# Autodesk Inventor assembly: ax4
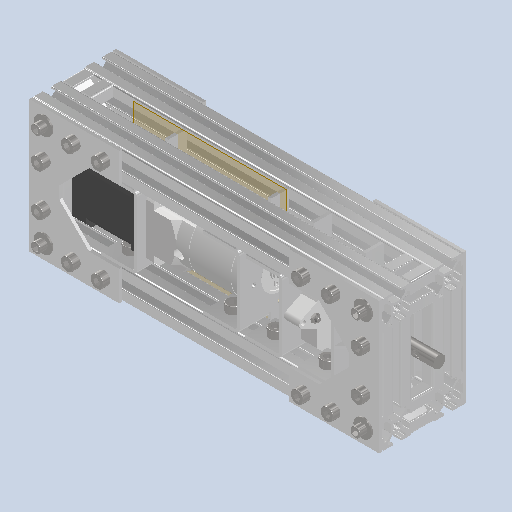
[picture p0: Inventor's stored thumbnail of the model, 512x512]
Saved by Autodesk Inventor 2024 (Build 280153000, 153)
## iProperties
Created: 2025-12-19
Part Number: ax4
Document SubType Name: Assembly
Designer: schar
Author: schar
## Documents named in this file (9)
- C:\Users\schar\Desktop\projectBlueprint\AMSTS\hardware\ax4.iam
- C:\Users\schar\Desktop\projectBlueprint\AMSTS\hardware\4x2020_in.iam
- C:\Users\schar\Desktop\projectBlueprint\AMSTS\hardware\4x2020_ax4.ipt
- C:\Users\schar\Desktop\projectBlueprint\AMSTS\hardware\2020_4x2020_hz.ipt
- C:\Users\schar\Desktop\projectBlueprint\AMSTS\hardware\2020_4x2020_ve.ipt
- C:\Users\schar\Desktop\projectBlueprint\AMSTS\hardware\Connect_u2020_asm.iam
- C:\Users\schar\Desktop\projectBlueprint\AMSTS\hardware\m4x70_example.ipt
- C:\Users\schar\Documents\Inventor\Content Center Files\R2024\en-US\DIN 9021\DIN 9021 - 4,3.ipt
- C:\Users\schar\Documents\Inventor\Content Center Files\R2024\en-US\ANSI B18.2.4.2M\ANSI B18.2.4.2M - M4x0,7 - 7.ipt
## Components (33 placed, 8 different names)
1. 4x2020_ax4:1 — Mate:1, Mate:2, Mate:3, Flush:1, Mate:4, Flush:2, Flush:4, Flush:8, Flush:10, Flush:13, Mate:12, Flush:17, Flush:18, Mate:15, Flush:23, Flush:24, Flush:28, Flush:31
2. 4x2020_ax4:2 — Mate:5, Flush:3, Flush:4, Flush:6, Mate:8, Flush:9, Mate:10, Flush:14, Mate:13, Flush:19, Flush:20, Mate:14, Flush:21, Flush:22, Mate:16, Flush:30
3. 4x2020_ax4:3 — Flush:7, Mate:7, Flush:8, Flush:11, Flush:12, Mate:11, Flush:15
4. 4x2020_ax4:4 — Mate:6, Flush:5, Flush:6, Mate:9, Flush:16, Flush:25, Flush:26
5. 4x2020_in:1 [sub-assembly] — Flush:1, Mate:4, Flush:2, Mate:5, Flush:3, Mate:6, Flush:5, Flush:7, Mate:7
6. 2020_4x2020_hz:1 — Mate:11, Flush:15, Flush:16
7. 2020_4x2020_hz:2 — Mate:10, Flush:13, Flush:14
8. 2020_4x2020_hz:3 — Mate:9, Flush:11, Flush:12
9. 2020_4x2020_hz:4 — Mate:8, Flush:9, Flush:10
10. 2020_4x2020_ve:1 — Mate:13, Flush:19, Flush:20, Flush:29, Mate:18
11. 2020_4x2020_ve:2 — Mate:12, Flush:17, Flush:18, Mate:19, Flush:32
12. 2020_4x2020_ve:3 — Mate:14, Flush:21, Flush:22
13. 2020_4x2020_ve:4 — Mate:15, Flush:23, Flush:24, Mate:17, Flush:27
14. Connect_u2020_asm:1 [sub-assembly] — Flush:25, Mate:16, Flush:26, Mate:22, Mate:23, Mate:24, Mate:25, Mate:40, Mate:42
15. Connect_u2020_asm:2 [sub-assembly] — Mate:17, Flush:27, Flush:28, Mate:20, Mate:21, Mate:26, Mate:27
16. Connect_u2020_asm:3 [sub-assembly] — Mate:19, Flush:31, Flush:32, Mate:28, Mate:29, Mate:30, Mate:31
17. Connect_u2020_asm:4 [sub-assembly] — Flush:29, Flush:30, Mate:18, Mate:32, Mate:33, Mate:34, Mate:35, Mate:36, Mate:38
18. m4x70_example:1 — Mate:42, Mate:43, Mate:48
19. m4x70_example:2 — Mate:40, Mate:41, Mate:50
20. m4x70_example:3 — Mate:38, Mate:39, Mate:46
21. m4x70_example:4 — Mate:36, Mate:37, Mate:44
22. DIN 9021 4,3:1 — Mate:32, Mate:35, Mate:37
23. DIN 9021 4,3:2 — Mate:24, Mate:25, Mate:43
24. DIN 9021 4,3:3 — Mate:22, Mate:23, Mate:41
25. DIN 9021 4,3:4 — Mate:33, Mate:34, Mate:39
26. DIN 9021 4,3:5 — Mate:20, Mate:21, Mate:51
27. DIN 9021 4,3:6 — Mate:26, Mate:27, Mate:49
28. DIN 9021 4,3:7 — Mate:30, Mate:31, Mate:45
29. DIN 9021 4,3:8 — Mate:28, Mate:29, Mate:47
30. ANSI B18.2.4.2M M4x0,7:1 — Mate:46, Mate:47
31. ANSI B18.2.4.2M M4x0,7:2 — Mate:48, Mate:49
32. ANSI B18.2.4.2M M4x0,7:3 — Mate:50, Mate:51
33. ANSI B18.2.4.2M M4x0,7:4 — Mate:44, Mate:45
## Relationships (83: Mate 51, Flush 32)
- Mate:1: 4x2020_ax4:1
- Mate:2: 4x2020_ax4:1
- Mate:3: 4x2020_ax4:1
- Flush:1 (20 mm): 4x2020_ax4:1 ↔ 4x2020_in:1
- Mate:4: 4x2020_ax4:1 ↔ 4x2020_in:1
- Flush:2: 4x2020_ax4:1 ↔ 4x2020_in:1
- Mate:5: 4x2020_ax4:2 ↔ 4x2020_in:1
- Flush:3: 4x2020_ax4:2 ↔ 4x2020_in:1
- Flush:4: 4x2020_ax4:1 ↔ 4x2020_ax4:2
- Mate:6: 4x2020_ax4:4 ↔ 4x2020_in:1
- Flush:5: 4x2020_ax4:4 ↔ 4x2020_in:1
- Flush:6: 4x2020_ax4:2 ↔ 4x2020_ax4:4
- Flush:7: 4x2020_ax4:3 ↔ 4x2020_in:1
- Mate:7: 4x2020_ax4:3 ↔ 4x2020_in:1
- Flush:8: 4x2020_ax4:1 ↔ 4x2020_ax4:3
- Mate:8: 4x2020_ax4:2 ↔ 2020_4x2020_hz:4
- Flush:9: 4x2020_ax4:2 ↔ 2020_4x2020_hz:4
- Flush:10: 4x2020_ax4:1 ↔ 2020_4x2020_hz:4
- Mate:9: 4x2020_ax4:4 ↔ 2020_4x2020_hz:3
- Flush:11: 4x2020_ax4:3 ↔ 2020_4x2020_hz:3
- Flush:12: 4x2020_ax4:3 ↔ 2020_4x2020_hz:3
- Mate:10: 4x2020_ax4:2 ↔ 2020_4x2020_hz:2
- Flush:13: 4x2020_ax4:1 ↔ 2020_4x2020_hz:2
- Flush:14: 4x2020_ax4:2 ↔ 2020_4x2020_hz:2
- Mate:11: 4x2020_ax4:3 ↔ 2020_4x2020_hz:1
- Flush:15: 4x2020_ax4:3 ↔ 2020_4x2020_hz:1
- Flush:16: 4x2020_ax4:4 ↔ 2020_4x2020_hz:1
- Mate:12: 4x2020_ax4:1 ↔ 2020_4x2020_ve:2
- Flush:17: 4x2020_ax4:1 ↔ 2020_4x2020_ve:2
- Flush:18: 4x2020_ax4:1 ↔ 2020_4x2020_ve:2
- Mate:13: 4x2020_ax4:2 ↔ 2020_4x2020_ve:1
- Flush:19: 4x2020_ax4:2 ↔ 2020_4x2020_ve:1
- Flush:20: 4x2020_ax4:2 ↔ 2020_4x2020_ve:1
- Mate:14: 4x2020_ax4:2 ↔ 2020_4x2020_ve:3
- Flush:21: 4x2020_ax4:2 ↔ 2020_4x2020_ve:3
- Flush:22: 4x2020_ax4:2 ↔ 2020_4x2020_ve:3
- Mate:15: 4x2020_ax4:1 ↔ 2020_4x2020_ve:4
- Flush:23: 4x2020_ax4:1 ↔ 2020_4x2020_ve:4
- Flush:24: 4x2020_ax4:1 ↔ 2020_4x2020_ve:4
- Flush:25: 4x2020_ax4:4 ↔ Connect_u2020_asm:1
- Mate:16: 4x2020_ax4:2 ↔ Connect_u2020_asm:1
- Flush:26: 4x2020_ax4:4 ↔ Connect_u2020_asm:1
- Mate:17: 2020_4x2020_ve:4 ↔ Connect_u2020_asm:2
- Flush:27: 2020_4x2020_ve:4 ↔ Connect_u2020_asm:2
- Flush:28: 4x2020_ax4:1 ↔ Connect_u2020_asm:2
- Flush:29: 2020_4x2020_ve:1 ↔ Connect_u2020_asm:4
- Flush:30: 4x2020_ax4:2 ↔ Connect_u2020_asm:4
- Mate:18: 2020_4x2020_ve:1 ↔ Connect_u2020_asm:4
- Mate:19: 2020_4x2020_ve:2 ↔ Connect_u2020_asm:3
- Flush:31: 4x2020_ax4:1 ↔ Connect_u2020_asm:3
- Flush:32: 2020_4x2020_ve:2 ↔ Connect_u2020_asm:3
- Mate:20: Connect_u2020_asm:2 ↔ DIN 9021 4,3:5
- Mate:21: Connect_u2020_asm:2 ↔ DIN 9021 4,3:5
- Mate:22: Connect_u2020_asm:1 ↔ DIN 9021 4,3:3
- Mate:23: Connect_u2020_asm:1 ↔ DIN 9021 4,3:3
- Mate:24: Connect_u2020_asm:1 ↔ DIN 9021 4,3:2
- Mate:25: Connect_u2020_asm:1 ↔ DIN 9021 4,3:2
- Mate:26: Connect_u2020_asm:2 ↔ DIN 9021 4,3:6
- Mate:27: Connect_u2020_asm:2 ↔ DIN 9021 4,3:6
- Mate:28: Connect_u2020_asm:3 ↔ DIN 9021 4,3:8
- Mate:29: Connect_u2020_asm:3 ↔ DIN 9021 4,3:8
- Mate:30: Connect_u2020_asm:3 ↔ DIN 9021 4,3:7
- Mate:31: Connect_u2020_asm:3 ↔ DIN 9021 4,3:7
- Mate:32: Connect_u2020_asm:4 ↔ DIN 9021 4,3:1
- Mate:33: Connect_u2020_asm:4 ↔ DIN 9021 4,3:4
- Mate:34: Connect_u2020_asm:4 ↔ DIN 9021 4,3:4
- Mate:35: Connect_u2020_asm:4 ↔ DIN 9021 4,3:1
- Mate:36: Connect_u2020_asm:4 ↔ m4x70_example:4
- Mate:37: m4x70_example:4 ↔ DIN 9021 4,3:1
- Mate:38: Connect_u2020_asm:4 ↔ m4x70_example:3
- Mate:39: m4x70_example:3 ↔ DIN 9021 4,3:4
- Mate:40: Connect_u2020_asm:1 ↔ m4x70_example:2
- Mate:41: m4x70_example:2 ↔ DIN 9021 4,3:3
- Mate:42: Connect_u2020_asm:1 ↔ m4x70_example:1
- Mate:43: m4x70_example:1 ↔ DIN 9021 4,3:2
- Mate:44: m4x70_example:4 ↔ ANSI B18.2.4.2M M4x0,7:4
- Mate:45: DIN 9021 4,3:7 ↔ ANSI B18.2.4.2M M4x0,7:4
- Mate:46: m4x70_example:3 ↔ ANSI B18.2.4.2M M4x0,7:1
- Mate:47: DIN 9021 4,3:8 ↔ ANSI B18.2.4.2M M4x0,7:1
- Mate:48: m4x70_example:1 ↔ ANSI B18.2.4.2M M4x0,7:2
- Mate:49: DIN 9021 4,3:6 ↔ ANSI B18.2.4.2M M4x0,7:2
- Mate:50: m4x70_example:2 ↔ ANSI B18.2.4.2M M4x0,7:3
- Mate:51: DIN 9021 4,3:5 ↔ ANSI B18.2.4.2M M4x0,7:3
